# Autodesk Inventor assembly: Alice
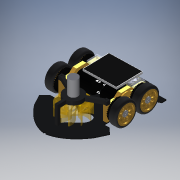
[picture p0: Inventor's stored thumbnail of the model, 180x180]
Saved by Autodesk Inventor 2016 (Build 200138000, 138)
## iProperties
Created: 2016-12-01
Part Number: Alice
Material: 一般
Document SubType Name: Weldment
Designer: KOTA-NPC2
Weld Material: Welded Aluminum-6061
Author: KOTA-NPC2
## Documents named in this file (7)
- C:\Users\B4_Ohno\Dropbox\AliCe関連\MicroMouse2016\Alice.iam
- C:\Users\B4_Ohno\Dropbox\AliCe関連\MicroMouse2016\AliCe_Motor.iam
- C:\Users\B4_Ohno\Dropbox\AliCe関連\MicroMouse2016\shitaita.ipt
- C:\Users\B4_Ohno\Dropbox\AliCe関連\MicroMouse2016\LiPo.ipt
- C:\Users\B4_Ohno\Dropbox\AliCe関連\MicroMouse2016\Assembly1.iam
- C:\Users\B4_Ohno\Dropbox\AliCe関連\MicroMouse2016\TFT_mount.ipt
- C:\Users\B4_Ohno\Dropbox\AliCe関連\MicroMouse2016\AliCe_TFT.iam
## Components (7 placed, 6 different names)
1. AliCe_Motor:1 [sub-assembly] — リジッド:1, 回転:1, 回転:4
2. AliCe_Motor:2 [sub-assembly] — リジッド:2, 回転:2, 回転:3
3. shitaita:1 — リジッド:1, リジッド:2, メイト:1
4. LiPo:1 — メイト:1
5. Assembly1:1 [sub-assembly] — 回転:1, 回転:2
6. TFT_mount:1 — 回転:3, 回転:4, 回転:5
7. AliCe_TFT:1 [sub-assembly] — 回転:5
## Relationships (8: RevoluteJoint 5, WeldJoint 2, Mate 1)
- リジッド:1 [WeldJoint]: AliCe_Motor:1 ↔ shitaita:1
- リジッド:2 [WeldJoint]: AliCe_Motor:2 ↔ shitaita:1
- 回転:1 [RevoluteJoint]: AliCe_Motor:1 ↔ Assembly1:1
- 回転:2 [RevoluteJoint]: AliCe_Motor:2 ↔ Assembly1:1
- 回転:3 [RevoluteJoint]: AliCe_Motor:2 ↔ TFT_mount:1
- 回転:4 [RevoluteJoint]: AliCe_Motor:1 ↔ TFT_mount:1
- メイト:1 [Mate]: shitaita:1 ↔ LiPo:1
- 回転:5 [RevoluteJoint]: TFT_mount:1 ↔ AliCe_TFT:1
